# Autodesk Inventor assembly: Full_Design_V1
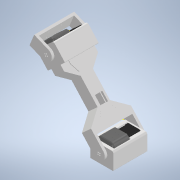
[picture p0: Inventor's stored thumbnail of the model, 180x180]
Saved by Autodesk Inventor 2022 (Build 260153000, 153)
## iProperties
Created: 2022-01-23
Part Number: Full_Design_V1
Document SubType Name: Assembly
Designer: Mlees
Author: Mlees
## Documents named in this file (17)
- C:\Users\Mlees\Desktop\504Engineering\Stepper-Servo_Based_Robotic_Arm\Designs\Version_4\Full_Design_V1.iam
- C:\Users\Mlees\Desktop\504Engineering\Stepper-Servo_Based_Robotic_Arm\Designs\Version_4\Created_Parts\96Gears_Stage_1.ipt
- C:\Users\Mlees\Desktop\504Engineering\Stepper-Servo_Based_Robotic_Arm\Designs\Version_4\Created_Parts\Nema17.ipt
- C:\Users\Mlees\Desktop\504Engineering\Stepper-Servo_Based_Robotic_Arm\Designs\Version_4\Created_Parts\96Gears_Stage_2.ipt
- C:\Users\Mlees\Desktop\504Engineering\Stepper-Servo_Based_Robotic_Arm\Designs\Version_4\Created_Parts\24_Teeth_Sun_Gear.ipt
- C:\Users\Mlees\Desktop\504Engineering\Stepper-Servo_Based_Robotic_Arm\Designs\Version_4\Created_Parts\36_Teeth_Planet_Gear.ipt
- C:\Users\Mlees\Desktop\504Engineering\Stepper-Servo_Based_Robotic_Arm\Designs\Version_4\Created_Parts\Planet_Carrier_Modifed_with_sun_gear.ipt
- C:\Users\Mlees\Desktop\504Engineering\Stepper-Servo_Based_Robotic_Arm\Designs\Version_4\Downloaded_Parts\nema17-speed-reducer-1.snapshot.9\Plamet_Carrier_modified.ipt
- C:\Users\Mlees\Desktop\504Engineering\Stepper-Servo_Based_Robotic_Arm\Designs\Version_4\Created_Parts\Gear_Cover_modified.ipt
- C:\Users\Mlees\Desktop\504Engineering\Stepper-Servo_Based_Robotic_Arm\Designs\Version_4\Created_Parts\Motor_Mount.ipt
- C:\Users\Mlees\Desktop\504Engineering\Stepper-Servo_Based_Robotic_Arm\Designs\Version_4\Created_Parts\Motor_Mount_Backplate.ipt
- C:\Users\Mlees\Desktop\504Engineering\Stepper-Servo_Based_Robotic_Arm\Designs\Version_4\Created_Parts\Bearing_mark_up.ipt
- C:\Users\Mlees\Desktop\504Engineering\Stepper-Servo_Based_Robotic_Arm\Designs\Version_4\Created_Parts\tilt_output_bracket.ipt
- C:\Users\Mlees\Desktop\504Engineering\Stepper-Servo_Based_Robotic_Arm\Designs\Version_4\Created_Parts\spacer.ipt
- C:\Users\Mlees\Desktop\504Engineering\Stepper-Servo_Based_Robotic_Arm\Designs\Version_4\Created_Parts\Tilt_Metal_Attachment.ipt
- C:\Users\Mlees\Desktop\504Engineering\Stepper-Servo_Based_Robotic_Arm\Designs\Version_4\Created_Parts\Metal_Bone.ipt
- C:\Users\Mlees\Desktop\504Engineering\Stepper-Servo_Based_Robotic_Arm\Designs\Version_4\Created_Parts\Metal_Shroud_tilt_1.ipt
## Components (42 placed, 16 different names)
1. 96Gears_Stage_1:1 — Rigid:1, Rigid:2
2. Nema17:1 — Rigid:1, Rotational:5, Rotational:6, Rigid:4
3. 96Gears_Stage_2:1 — Rigid:2, Rigid:3
4. 24_Teeth_Sun_Gear:1 — Rotational:5
5. 36_Teeth_Planet_Gear:1 — Rotational:4
6. 36_Teeth_Planet_Gear:2 — Rotational:2
7. 36_Teeth_Planet_Gear:3 — Rotational:3
8. Planet_Carrier_Modifed_with_sun_gear:1 — Rotational:2, Rotational:3, Rotational:4, Rotational:6, Rotational:10
9. Plamet_Carrier_modified:1 — Rotational:7, Rotational:8, Rotational:9, Rotational:10, Rotational:11, Rotational:13
10. 36_Teeth_Planet_Gear:4 — Rotational:7
11. 36_Teeth_Planet_Gear:5 — Rotational:9
12. 36_Teeth_Planet_Gear:6 — Rotational:8
13. Gear_Cover_modified:1 — Rigid:3
14. Motor_Mount:1 — Rigid:4, Rigid:5
15. Motor_Mount_Backplate:1 — Rigid:5, Rotational:12
16. Bearing_mark_up:1 — Rotational:12
17. Bearing_mark_up:2 — Rotational:11
18. tilt_output_bracket:1 — Rigid:6, Rigid:7
19. spacer:1 — Rigid:6, Rotational:13
20. Tilt_Metal_Attachment:1 — Rigid:7, Rigid:8, Rigid:11
21. Metal_Bone:1 — Rigid:8, Rigid:9
22. Tilt_Metal_Attachment:2 — Rigid:9, Rigid:10
23. Motor_Mount:2 — Rigid:10, Rigid:18, Rotational:17, Rigid:20
24. Metal_Shroud_tilt_1:1 — Rigid:11
25. Nema17:2 — Rigid:12, Rotational:14, Rotational:15, Rigid:20
26. tilt_output_bracket:2 — Rotational:23
27. Motor_Mount_Backplate:2 — Rigid:18, Rotational:16
28. Gear_Cover_modified:2 — Rigid:19
29. Bearing_mark_up:3 — Rotational:16, Rotational:23
30. Bearing_mark_up:4 — Rotational:17
31. 96Gears_Stage_2:2 — Rigid:13, Rigid:19
32. 96Gears_Stage_1:2 — Rigid:12, Rigid:13
33. 36_Teeth_Planet_Gear:7 — Rigid:14
34. 36_Teeth_Planet_Gear:8 — Rigid:15
35. 36_Teeth_Planet_Gear:9 — Rigid:16
36. 36_Teeth_Planet_Gear:10 — Rotational:18
37. 36_Teeth_Planet_Gear:11 — Rotational:19
38. 36_Teeth_Planet_Gear:12 — Rotational:20
39. 24_Teeth_Sun_Gear:2 — Rotational:14
40. Planet_Carrier_Modifed_with_sun_gear:2 — Rigid:14, Rigid:15, Rigid:16, Rotational:15, Rotational:21
41. Plamet_Carrier_modified:2 — Rotational:18, Rotational:19, Rotational:20, Rotational:21, Rotational:22
42. spacer:2 — Rotational:22
## Relationships (41: RevoluteJoint 22, WeldJoint 19)
- Rigid:1 [WeldJoint]: 96Gears_Stage_1:1 ↔ Nema17:1
- Rigid:2 [WeldJoint]: 96Gears_Stage_1:1 ↔ 96Gears_Stage_2:1
- Rotational:2 [RevoluteJoint]: 36_Teeth_Planet_Gear:2 ↔ Planet_Carrier_Modifed_with_sun_gear:1
- Rotational:3 [RevoluteJoint]: 36_Teeth_Planet_Gear:3 ↔ Planet_Carrier_Modifed_with_sun_gear:1
- Rotational:4 [RevoluteJoint]: 36_Teeth_Planet_Gear:1 ↔ Planet_Carrier_Modifed_with_sun_gear:1
- Rotational:5 [RevoluteJoint]: Nema17:1 ↔ 24_Teeth_Sun_Gear:1
- Rotational:6 [RevoluteJoint]: Nema17:1 ↔ Planet_Carrier_Modifed_with_sun_gear:1
- Rotational:7 [RevoluteJoint]: Plamet_Carrier_modified:1 ↔ 36_Teeth_Planet_Gear:4
- Rotational:8 [RevoluteJoint]: Plamet_Carrier_modified:1 ↔ 36_Teeth_Planet_Gear:6
- Rotational:9 [RevoluteJoint]: Plamet_Carrier_modified:1 ↔ 36_Teeth_Planet_Gear:5
- Rotational:10 [RevoluteJoint]: Planet_Carrier_Modifed_with_sun_gear:1 ↔ Plamet_Carrier_modified:1
- Rigid:3 [WeldJoint]: 96Gears_Stage_2:1 ↔ Gear_Cover_modified:1
- Rigid:4 [WeldJoint] (1 mm): Nema17:1 ↔ Motor_Mount:1
- Rigid:5 [WeldJoint]: Motor_Mount:1 ↔ Motor_Mount_Backplate:1
- Rotational:11 [RevoluteJoint]: Plamet_Carrier_modified:1 ↔ Bearing_mark_up:2
- Rotational:12 [RevoluteJoint]: Motor_Mount_Backplate:1 ↔ Bearing_mark_up:1
- Rigid:6 [WeldJoint]: tilt_output_bracket:1 ↔ spacer:1
- Rotational:13 [RevoluteJoint]: Plamet_Carrier_modified:1 ↔ spacer:1
- Rigid:7 [WeldJoint]: tilt_output_bracket:1 ↔ Tilt_Metal_Attachment:1
- Rigid:8 [WeldJoint]: Tilt_Metal_Attachment:1 ↔ Metal_Bone:1
- Rigid:9 [WeldJoint]: Metal_Bone:1 ↔ Tilt_Metal_Attachment:2
- Rigid:10 [WeldJoint]: Tilt_Metal_Attachment:2 ↔ Motor_Mount:2
- Rigid:11 [WeldJoint]: Tilt_Metal_Attachment:1 ↔ Metal_Shroud_tilt_1:1
- Rigid:12 [WeldJoint]: Nema17:2 ↔ 96Gears_Stage_1:2
- Rigid:13 [WeldJoint]: 96Gears_Stage_2:2 ↔ 96Gears_Stage_1:2
- Rigid:14 [WeldJoint]: 36_Teeth_Planet_Gear:7 ↔ Planet_Carrier_Modifed_with_sun_gear:2
- Rigid:15 [WeldJoint]: 36_Teeth_Planet_Gear:8 ↔ Planet_Carrier_Modifed_with_sun_gear:2
- Rigid:16 [WeldJoint]: 36_Teeth_Planet_Gear:9 ↔ Planet_Carrier_Modifed_with_sun_gear:2
- Rotational:14 [RevoluteJoint]: Nema17:2 ↔ 24_Teeth_Sun_Gear:2
- Rotational:15 [RevoluteJoint]: Nema17:2 ↔ Planet_Carrier_Modifed_with_sun_gear:2
- Rigid:18 [WeldJoint]: Motor_Mount:2 ↔ Motor_Mount_Backplate:2
- Rotational:16 [RevoluteJoint]: Motor_Mount_Backplate:2 ↔ Bearing_mark_up:3
- Rotational:17 [RevoluteJoint]: Motor_Mount:2 ↔ Bearing_mark_up:4
- Rotational:18 [RevoluteJoint]: 36_Teeth_Planet_Gear:10 ↔ Plamet_Carrier_modified:2
- Rotational:19 [RevoluteJoint]: 36_Teeth_Planet_Gear:11 ↔ Plamet_Carrier_modified:2
- Rotational:20 [RevoluteJoint]: 36_Teeth_Planet_Gear:12 ↔ Plamet_Carrier_modified:2
- Rotational:21 [RevoluteJoint]: Planet_Carrier_Modifed_with_sun_gear:2 ↔ Plamet_Carrier_modified:2
- Rigid:19 [WeldJoint]: Gear_Cover_modified:2 ↔ 96Gears_Stage_2:2
- Rigid:20 [WeldJoint] (1 mm): Motor_Mount:2 ↔ Nema17:2
- Rotational:22 [RevoluteJoint]: Plamet_Carrier_modified:2 ↔ spacer:2
- Rotational:23 [RevoluteJoint] (-2.5 mm): tilt_output_bracket:2 ↔ Bearing_mark_up:3
